# Autodesk Inventor assembly: Fr.wing_assy
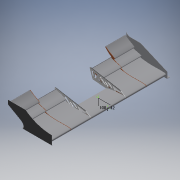
[picture p0: Inventor's stored thumbnail of the model, 180x180]
Saved by Autodesk Inventor 2018 (Build 220112000, 112)
## iProperties
Created: 2018-03-05
Part Number: Fr.wing_assy
Material: 一般
Document SubType Name: Assembly
Designer: ku_sk
Mass: 11232.8 g
Surface Area: 27769.7 cm^2
Volume: 11454.5 cm^3
Density: 0.980642 g/cm^3
Author: ku_sk
## Documents named in this file (11)
- D:\Users\ku_sk\Documents\Inventor\Aero\KS-15\Fr.wing\Fr.wing_assy.iam
- D:\Users\ku_sk\Documents\Inventor\Aero\KS-15\Fr.wing\parts\mainflap_side\mainflap_side.iam
- D:\Users\ku_sk\Documents\Inventor\Aero\KS-15\Fr.wing\parts\mainflap_center\mainflap_center.iam
- D:\Users\ku_sk\Documents\Inventor\Aero\KS-15\Fr.wing\parts\subflap\subflap.iam
- D:\Users\ku_sk\Documents\Inventor\Aero\KS-15\Fr.wing\parts\bracket1\bracket1.ipt
- D:\Users\ku_sk\Documents\Inventor\Aero\KS-15\Fr.wing\parts\bracket2.ipt
- D:\Users\ku_sk\Documents\Inventor\Aero\KS-15\Fr.wing\parts\endplate1.ipt
- D:\Users\ku_sk\Documents\Inventor\Aero\KS-15\Fr.wing\parts\axis_f3.ipt
- D:\Users\ku_sk\Documents\Inventor\Aero\KS-15\Fr.wing\parts\axis_f2.ipt
- D:\Users\ku_sk\Documents\Inventor\Aero\KS-15\Fr.wing\parts\axis_f1.ipt
- D:\Users\ku_sk\Documents\Inventor\Aero\KS-15\Fr.wing\parts\endplate_ver2.ipt
## Components (27 placed, 10 different names)
1. mainflap_center:1 [sub-assembly] — フラッシュ:1, メイト:1, メイト:4, メイト:5, メイト:6, メイト:7, 角度:1, メイト:50, メイト:51, メイト:52, メイト:53, メイト:54, メイト:55
2. mainflap_side:1 [sub-assembly] — メイト:4, メイト:7, メイト:8, メイト:9, メイト:10, フラッシュ:2, メイト:46, メイト:56, メイト:57, メイト:64
3. mainflap_side:2 [sub-assembly] — メイト:5, メイト:6, メイト:11, メイト:12, メイト:13, フラッシュ:4, メイト:49, メイト:65
4. mainflap_side:3 [sub-assembly] — メイト:8, メイト:9, メイト:10, フラッシュ:3, メイト:45, メイト:78, メイト:79, フラッシュ:20
5. mainflap_side:4 [sub-assembly] — メイト:11, メイト:12, メイト:13, フラッシュ:5, メイト:80
6. subflap:1 [sub-assembly] — メイト:14, メイト:15, メイト:19, フラッシュ:2, メイト:20, メイト:21, メイト:58, メイト:59
7. subflap:2 [sub-assembly] — メイト:14, メイト:15, メイト:19, フラッシュ:3, フラッシュ:7
8. subflap:3 [sub-assembly] — メイト:22, メイト:23, フラッシュ:7, メイト:60, メイト:61
9. subflap:4 [sub-assembly] — メイト:16, メイト:17, メイト:18, フラッシュ:4, メイト:20, メイト:21, メイト:63
10. subflap:5 [sub-assembly] — メイト:16, メイト:17, メイト:18, フラッシュ:5, フラッシュ:6, メイト:76, フラッシュ:18, メイト:77
11. subflap:6 [sub-assembly] — メイト:22, メイト:23, フラッシュ:6, メイト:62
12. bracket2:1 — メイト:46, メイト:56, メイト:57, メイト:58, メイト:59, メイト:60, メイト:61, メイト:72, メイト:73, フラッシュ:14
13. bracket2:2 — メイト:49, メイト:62, メイト:63, メイト:70, メイト:71, フラッシュ:12
14. bracket1:1 — メイト:52, メイト:53, メイト:54, メイト:65
15. bracket1:2 — メイト:50, メイト:51, メイト:55, メイト:64, メイト:74, メイト:75, フラッシュ:16
16. axis_f3:1 — フラッシュ:11, メイト:71
17. axis_f3:2 — フラッシュ:11, メイト:70, フラッシュ:12
18. axis_f3:3 — フラッシュ:13, メイト:73
19. axis_f3:4 — フラッシュ:13, メイト:72, フラッシュ:14
20. axis_f2:1 — フラッシュ:17, メイト:77
21. axis_f2:2 — フラッシュ:17, メイト:76, フラッシュ:18
22. axis_f2:3 — フラッシュ:15, メイト:75, フラッシュ:16
23. axis_f2:4 — フラッシュ:15, メイト:74
24. axis_f1:1 — フラッシュ:19, メイト:79
25. axis_f1:2 — フラッシュ:19, メイト:78, フラッシュ:20
26. endplate1:1 — メイト:45, フラッシュ:21, フラッシュ:22, フラッシュ:23
27. endplate_ver2:1 — メイト:80, フラッシュ:21, フラッシュ:22, メイト:81
## Relationships (73: Mate 52, Flush 20, Angle 1)
- フラッシュ:1 [Flush]: mainflap_center:1
- メイト:1 [Mate]: mainflap_center:1
- メイト:4 [Mate]: mainflap_center:1 ↔ mainflap_side:1
- メイト:5 [Mate]: mainflap_center:1 ↔ mainflap_side:2
- メイト:6 [Mate]: mainflap_center:1 ↔ mainflap_side:2
- メイト:7 [Mate]: mainflap_center:1 ↔ mainflap_side:1
- メイト:8 [Mate] (4 mm): mainflap_side:1 ↔ mainflap_side:3
- メイト:9 [Mate]: mainflap_side:1 ↔ mainflap_side:3
- メイト:10 [Mate]: mainflap_side:1 ↔ mainflap_side:3
- メイト:11 [Mate] (4 mm): mainflap_side:2 ↔ mainflap_side:4
- メイト:12 [Mate]: mainflap_side:2 ↔ mainflap_side:4
- メイト:13 [Mate]: mainflap_side:2 ↔ mainflap_side:4
- メイト:14 [Mate]: subflap:1 ↔ subflap:2
- メイト:15 [Mate]: subflap:1 ↔ subflap:2
- メイト:16 [Mate] (4 mm): subflap:4 ↔ subflap:5
- メイト:17 [Mate]: subflap:4 ↔ subflap:5
- メイト:18 [Mate]: subflap:4 ↔ subflap:5
- メイト:19 [Mate] (4 mm): subflap:1 ↔ subflap:2
- フラッシュ:2 [Flush]: mainflap_side:1 ↔ subflap:1
- フラッシュ:3 [Flush]: mainflap_side:3 ↔ subflap:2
- フラッシュ:4 [Flush]: mainflap_side:2 ↔ subflap:4
- フラッシュ:5 [Flush]: mainflap_side:4 ↔ subflap:5
- メイト:20 [Mate]: subflap:1 ↔ subflap:4
- メイト:21 [Mate]: subflap:1 ↔ subflap:4
- メイト:22 [Mate]: subflap:3 ↔ subflap:6
- メイト:23 [Mate]: subflap:3 ↔ subflap:6
- フラッシュ:6 [Flush]: subflap:5 ↔ subflap:6
- フラッシュ:7 [Flush]: subflap:2 ↔ subflap:3
- メイト:45 [Mate]: mainflap_side:3 ↔ endplate1:1
- 角度:1 [Angle] (4 deg): mainflap_center:1
- メイト:46 [Mate]: mainflap_side:1 ↔ bracket2:1
- メイト:49 [Mate]: mainflap_side:2 ↔ bracket2:2
- メイト:50 [Mate]: mainflap_center:1 ↔ bracket1:2
- メイト:51 [Mate]: mainflap_center:1 ↔ bracket1:2
- メイト:52 [Mate]: mainflap_center:1 ↔ bracket1:1
- メイト:53 [Mate]: mainflap_center:1 ↔ bracket1:1
- メイト:54 [Mate]: mainflap_center:1 ↔ bracket1:1
- メイト:55 [Mate]: mainflap_center:1 ↔ bracket1:2
- メイト:56 [Mate]: mainflap_side:1 ↔ bracket2:1
- メイト:57 [Mate]: mainflap_side:1 ↔ bracket2:1
- メイト:58 [Mate]: subflap:1 ↔ bracket2:1
- メイト:59 [Mate]: subflap:1 ↔ bracket2:1
- メイト:60 [Mate]: subflap:3 ↔ bracket2:1
- メイト:61 [Mate]: subflap:3 ↔ bracket2:1
- メイト:62 [Mate]: subflap:6 ↔ bracket2:2
- メイト:63 [Mate]: subflap:4 ↔ bracket2:2
- メイト:64 [Mate]: mainflap_side:1 ↔ bracket1:2
- メイト:65 [Mate]: mainflap_side:2 ↔ bracket1:1
- フラッシュ:11 [Flush]: axis_f3:1 ↔ axis_f3:2
- メイト:70 [Mate]: bracket2:2 ↔ axis_f3:2
- メイト:71 [Mate]: bracket2:2 ↔ axis_f3:1
- フラッシュ:12 [Flush]: bracket2:2 ↔ axis_f3:2
- フラッシュ:13 [Flush]: axis_f3:3 ↔ axis_f3:4
- メイト:72 [Mate]: bracket2:1 ↔ axis_f3:4
- メイト:73 [Mate]: bracket2:1 ↔ axis_f3:3
- フラッシュ:14 [Flush]: bracket2:1 ↔ axis_f3:4
- フラッシュ:15 [Flush]: axis_f2:3 ↔ axis_f2:4
- メイト:74 [Mate]: bracket1:2 ↔ axis_f2:4
- メイト:75 [Mate]: bracket1:2 ↔ axis_f2:3
- フラッシュ:16 [Flush]: bracket1:2 ↔ axis_f2:3
- フラッシュ:17 [Flush]: axis_f2:1 ↔ axis_f2:2
- メイト:76 [Mate]: subflap:5 ↔ axis_f2:2
- フラッシュ:18 [Flush]: subflap:5 ↔ axis_f2:2
- メイト:77 [Mate]: subflap:5 ↔ axis_f2:1
- フラッシュ:19 [Flush]: axis_f1:1 ↔ axis_f1:2
- メイト:78 [Mate]: mainflap_side:3 ↔ axis_f1:2
- メイト:79 [Mate]: mainflap_side:3 ↔ axis_f1:1
- フラッシュ:20 [Flush]: mainflap_side:3 ↔ axis_f1:2
- メイト:80 [Mate]: mainflap_side:4 ↔ endplate_ver2:1
- フラッシュ:21 [Flush]: endplate1:1 ↔ endplate_ver2:1
- フラッシュ:22 [Flush]: endplate1:1 ↔ endplate_ver2:1
- フラッシュ:23 [Flush] (-20 mm): endplate1:1
- メイト:81 [Mate] (-32 mm): endplate_ver2:1
